# Autodesk Inventor assembly: Araknid-4Wire-Laser-Slot-x4
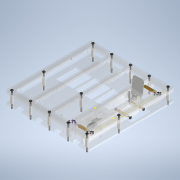
[picture p0: Inventor's stored thumbnail of the model, 180x180]
Saved by Autodesk Inventor 2021 (Build 250183000, 183)
## iProperties
Created: 2020-06-23
Part Number: Araknid-4Wire-Laser-Slot-x4
Document SubType Name: Assembly
Designer: lucas
Project: 4Wire-Laser
Author: lucas
Revision Number: RLS_001
## Documents named in this file (22)
- C:\Users\lucas\Nextcloud\HackerSpace\HV Home Battery Storage Project\Concepts & Storyboards\18650 4wire Holder\Araknid-4Wire-Laser-Slot-x4.iam
- C:\Users\lucas\Nextcloud\HackerSpace\HV Home Battery Storage Project\Concepts & Storyboards\18650 4wire Holder\4Wire-Laser-Slot\Laser-Slot-Term-Beam.ipt
- C:\Users\lucas\Nextcloud\HackerSpace\HV Home Battery Storage Project\Concepts & Storyboards\18650 4wire Holder\4Wire-Laser-Slot\Laser-Slot-Side.ipt
- C:\Users\lucas\Nextcloud\HackerSpace\HV Home Battery Storage Project\Concepts & Storyboards\18650 4wire Holder\4Wire-Laser-Slot\Laser-Slot-Bottom.ipt
- C:\Users\lucas\Nextcloud\HackerSpace\HV Home Battery Storage Project\Concepts & Storyboards\18650 4wire Holder\4Wire-Laser-Slot\Laser-Pivot-Term-Beam.ipt
- C:\Users\lucas\Nextcloud\HackerSpace\HV Home Battery Storage Project\Concepts & Storyboards\18650 4wire Holder\4Wire-Laser-Slot\Laser-Pivot-Side.ipt
- C:\Users\lucas\Nextcloud\HackerSpace\HV Home Battery Storage Project\Concepts & Storyboards\18650 4wire Holder\4Wire-Laser-Slot\Laser-Slot-Side_Mirror.ipt
- C:\Users\lucas\Nextcloud\HackerSpace\HV Home Battery Storage Project\Concepts & Storyboards\18650 4wire Holder\4Wire-Laser-Slot\Standoff-M3x26mm.ipt
- C:\Users\lucas\Nextcloud\HackerSpace\HV Home Battery Storage Project\Concepts & Storyboards\18650 4wire Holder\4Wire-Laser-Slot\Shaft5.ipt
- C:\Users\lucas\Nextcloud\HackerSpace\HV Home Battery Storage Project\Concepts & Storyboards\18650 4wire Holder\4Wire-Laser-Slot\Standoff-M3x20mm.ipt
- C:\Users\lucas\Nextcloud\HackerSpace\HV Home Battery Storage Project\Concepts & Storyboards\18650 4wire Holder\4Wire-Laser-Slot\Shaft7.ipt
- C:\Users\lucas\Nextcloud\HackerSpace\HV Home Battery Storage Project\Concepts & Storyboards\18650 4wire Holder\ZKE\ZKE-Term-Solid.ipt
- C:\Users\lucas\Nextcloud\HackerSpace\HV Home Battery Storage Project\Concepts & Storyboards\18650 4wire Holder\4Wire-Laser-Slot\Laser-Base-x4.ipt
- C:\Users\lucas\Nextcloud\HackerSpace\HV Home Battery Storage Project\Concepts & Storyboards\18650 4wire Holder\4Wire-Laser-Slot\Laser-Pivot-Ringpull.ipt
- C:\Users\lucas\Nextcloud\HackerSpace\HV Home Battery Storage Project\Concepts & Storyboards\18650 4wire Holder\4Wire-Laser-Slot\Laser-Slot-Endstop.ipt
- C:\Users\lucas\Nextcloud\HackerSpace\HV Home Battery Storage Project\Concepts & Storyboards\18650 4wire Holder\ZKE\ZKE-Term-Sprung.ipt
- C:\Users\lucas\Nextcloud\HackerSpace\HV Home Battery Storage Project\Concepts & Storyboards\18650 4wire Holder\ZKE\ZKE-Term-Solid-Shim.ipt
- C:\Users\lucas\Nextcloud\HackerSpace\HV Home Battery Storage Project\Concepts & Storyboards\18650 4wire Holder\4Wire-Laser-Slot\Laser-Slot-Top.ipt
- C:\Users\lucas\Nextcloud\HackerSpace\HV Home Battery Storage Project\Concepts & Storyboards\18650 4wire Holder\4Wire-Laser-Slot\Standoff-TH-M3x17mm.ipt
- C:\Users\lucas\Documents\Inventor\Content Center Files\R2021\en-US\ISO 7380-1\ISO 7380-1 - M3 x 10.ipt
- C:\Users\lucas\Documents\Inventor\Content Center Files\R2021\en-US\ISO 7380-1\ISO 7380-1 - M3 x 12.ipt
- C:\Users\lucas\Documents\Inventor\Content Center Files\R2021\en-US\ISO 4762(2)\ISO 4762 - M3 x 10ISO.ipt
## Components (52 placed, 17 different names)
1. PosTerminalBeamr:1 — Mate:24, Flush:6, Flush:10, Mate:38, Mate:39, Rotational:3
2. Laser-Slot-Side:2 — Flush:1, Mate:24, Flush:6, Mate:27, Flush:8, Mate:34, Mate:35, Flush:11, Flush:12, Mate:46, Mate:47, Flush:17, Mate:49, Mate:52, Mate:53
3. Laser-Slot-Endstop:1 — Mate:46, Mate:47, Flush:17
4. Laser-Slot-Bottom:1 — Mate:51, Mate:52, Mate:53
5. ZKE-Term-Sprung:1 — Rotational:3
6. Laser-Pivot-Term-Beam:1 — Mate:6, Mate:10, Flush:2, Flush:3, Mate:48, Rotational:5, Rotational:6, Rotational:7
7. Laser-Pivot-Side:1 — Mate:10, Flush:2, Mate:44, Flush:13, Angle:4, Mate:45, Flush:14, Angle:5, Flush:16
8. Laser-Pivot-Side:2 — Mate:6, Flush:3, Rotational:4, Rotation:1, Flush:16, Mate:48
9. Laser-Slot-Side_Mirror:1 — Mate:4, Mate:26, Flush:7, Mate:32, Mate:33, Flush:10, Mate:38, Mate:39, Flush:11, Flush:12, Rotational:1, Rotation:1, Mate:50, Mate:51
10. Shaft:1 — Mate:44, Flush:13, Angle:4
11. Shaft:1 — Mate:45, Flush:14, Angle:5
12. ISO 4762 M3 x 10:1
13. ISO 4762 M3 x 10:2
14. ISO 7380-1 M3 x 10:3
15. ISO 7380-1 M3 x 10:4
16. Shaft:1 — Mate:26, Flush:7
17. Shaft:1 — Mate:27, Flush:8
18. ISO 4762 M3 x 10:3
19. ISO 4762 M3 x 10:4
20. ISO 7380-1 M3 x 10:1 — Mate:32, Mate:33
21. ISO 7380-1 M3 x 10:2 — Mate:34, Mate:35
22. ZKE-Term-Solid:1 — Rotational:7
23. Laser-Base-x4:1 — Rotational:1, Rotational:4, Rotational:8, Rotational:9, Rotational:10, Rotational:11, Rigid:1, Rotational:12, Rotational:13, Rotational:14, Rotational:15, Rotational:16, Rotational:17, Rigid:2, Rotational:18, Mate:54, Mate:55, Mate:56, Mate:57, Mate:58, Mate:59, Mate:60, Mate:61, Mate:62, Mate:63, Mate:64, Mate:65, Mate:66, Mate:67, Mate:68, Mate:69, Mate:70, Mate:71, Mate:72, Mate:73, Mate:74, Mate:75, Mate:76, Mate:77, Mate:78, Mate:79
24. Laser-Pivot-Ringpull:1 — Rotational:5
25. ZKE-Term-Solid-Shim:1 — Rotational:6
26. Laser-Slot-Top:1 — Mate:49, Mate:50
27. Shaft:1 — Rotational:8
28. Shaft:2 — Rotational:10
29. Shaft:3 — Rotational:9
30. Shaft:4 — Rotational:11
31. Shaft:5 — Rigid:1
32. Shaft:6 — Rotational:16
33. Shaft:7 — Rotational:14
34. Shaft:8 — Rotational:15
35. Shaft:9 — Rotational:13
36. Shaft:10 — Rotational:12
37. Shaft:11 — Rotational:18
38. Shaft:12 — Rigid:2
39. Shaft:13 — Rotational:17
40. ISO 7380-1 M3 x 12:3 — Mate:54, Mate:55
41. ISO 7380-1 M3 x 12:4 — Mate:56, Mate:57
42. ISO 7380-1 M3 x 12:5 — Mate:58, Mate:59
43. ISO 7380-1 M3 x 12:6 — Mate:60, Mate:61
44. ISO 7380-1 M3 x 12:7 — Mate:62, Mate:63
45. ISO 7380-1 M3 x 12:8 — Mate:64, Mate:65
46. ISO 7380-1 M3 x 12:9 — Mate:66, Mate:67
47. ISO 7380-1 M3 x 12:10 — Mate:68, Mate:69
48. ISO 7380-1 M3 x 12:11 — Mate:70, Mate:71
49. ISO 7380-1 M3 x 12:12 — Mate:72, Mate:73
50. ISO 7380-1 M3 x 12:13 — Mate:74, Mate:75
51. ISO 7380-1 M3 x 12:14 — Mate:76, Mate:77
52. ISO 7380-1 M3 x 12:15 — Mate:78, Mate:79
## Relationships (95: Mate 60, RevoluteJoint 17, Flush 13, Angle 2, WeldJoint 2, RelateRotation 1)
- Flush:1 (10 mm): Laser-Slot-Side:2
- Mate:4 (10 mm): Laser-Slot-Side_Mirror:1
- Mate:6 (0.075 mm): Laser-Pivot-Term-Beam:1 ↔ Laser-Pivot-Side:2
- Mate:10 (0.075 mm): Laser-Pivot-Term-Beam:1 ↔ Laser-Pivot-Side:1
- Flush:2: Laser-Pivot-Term-Beam:1 ↔ Laser-Pivot-Side:1
- Flush:3: Laser-Pivot-Term-Beam:1 ↔ Laser-Pivot-Side:2
- [Mate]: Shaft:1 ↔ ISO 4762 M3 x 10:1
- [Mate]: Laser-Pivot-Side:1 ↔ ISO 4762 M3 x 10:1
- [Mate]: Shaft:1 ↔ ISO 4762 M3 x 10:2
- [Mate]: Laser-Pivot-Side:2 ↔ ISO 4762 M3 x 10:2
- [Mate]: Laser-Pivot-Side:1 ↔ ISO 7380-1 M3 x 10:3
- [Mate]: Laser-Pivot-Side:1 ↔ ISO 7380-1 M3 x 10:3
- [Mate]: Laser-Pivot-Side:2 ↔ ISO 7380-1 M3 x 10:4
- [Mate]: Laser-Pivot-Side:2 ↔ ISO 7380-1 M3 x 10:4
- Mate:24 (0.075 mm): PosTerminalBeamr:1 ↔ Laser-Slot-Side:2
- Flush:6: PosTerminalBeamr:1 ↔ Laser-Slot-Side:2
- Mate:26: Laser-Slot-Side_Mirror:1 ↔ Shaft:1
- Flush:7: Laser-Slot-Side_Mirror:1 ↔ Shaft:1
- Mate:27: Laser-Slot-Side:2 ↔ Shaft:1
- Flush:8: Laser-Slot-Side:2 ↔ Shaft:1
- [Mate]: Laser-Slot-Side:2 ↔ ISO 4762 M3 x 10:3
- [Mate]: Laser-Slot-Side:2 ↔ ISO 4762 M3 x 10:3
- [Mate]: Laser-Slot-Side_Mirror:1 ↔ ISO 4762 M3 x 10:4
- [Mate]: Laser-Slot-Side_Mirror:1 ↔ ISO 4762 M3 x 10:4
- Mate:32: Laser-Slot-Side_Mirror:1 ↔ ISO 7380-1 M3 x 10:1
- Mate:33: Laser-Slot-Side_Mirror:1 ↔ ISO 7380-1 M3 x 10:1
- Mate:34: Laser-Slot-Side:2 ↔ ISO 7380-1 M3 x 10:2
- Mate:35: Laser-Slot-Side:2 ↔ ISO 7380-1 M3 x 10:2
- Rotational:1 [RevoluteJoint] (1 mm): Laser-Slot-Side_Mirror:1 ↔ Laser-Base-x4:1
- Flush:10: PosTerminalBeamr:1 ↔ Laser-Slot-Side_Mirror:1
- Mate:38 (0.075 mm): PosTerminalBeamr:1 ↔ Laser-Slot-Side_Mirror:1
- Mate:39 (0.075 mm): PosTerminalBeamr:1 ↔ Laser-Slot-Side_Mirror:1
- Flush:11: Laser-Slot-Side:2 ↔ Laser-Slot-Side_Mirror:1
- Flush:12: Laser-Slot-Side:2 ↔ Laser-Slot-Side_Mirror:1
- Rotational:3 [RevoluteJoint]: PosTerminalBeamr:1 ↔ ZKE-Term-Sprung:1
- Rotational:4 [RevoluteJoint] (1 mm): Laser-Pivot-Side:2 ↔ Laser-Base-x4:1
- Rotation:1 [RelateRotation] (2.55 ul): Laser-Pivot-Side:2 ↔ Laser-Slot-Side_Mirror:1
- Mate:44: Laser-Pivot-Side:1 ↔ Shaft:1
- Flush:13: Laser-Pivot-Side:1 ↔ Shaft:1
- Angle:4 (0 deg): Laser-Pivot-Side:1 ↔ Shaft:1
- Mate:45: Laser-Pivot-Side:1 ↔ Shaft:1
- Flush:14: Laser-Pivot-Side:1 ↔ Shaft:1
- Angle:5 (0 deg): Laser-Pivot-Side:1 ↔ Shaft:1
- Mate:46: Laser-Slot-Side:2 ↔ Laser-Slot-Endstop:1
- Mate:47: Laser-Slot-Side:2 ↔ Laser-Slot-Endstop:1
- Flush:16: Laser-Pivot-Side:1 ↔ Laser-Pivot-Side:2
- Mate:48: Laser-Pivot-Term-Beam:1 ↔ Laser-Pivot-Side:2
- Flush:17 (2.75 mm): Laser-Slot-Side:2 ↔ Laser-Slot-Endstop:1
- Rotational:5 [RevoluteJoint]: Laser-Pivot-Term-Beam:1 ↔ Laser-Pivot-Ringpull:1
- Rotational:6 [RevoluteJoint]: Laser-Pivot-Term-Beam:1 ↔ ZKE-Term-Solid-Shim:1
- Rotational:7 [RevoluteJoint]: Laser-Pivot-Term-Beam:1 ↔ ZKE-Term-Solid:1
- Mate:49: Laser-Slot-Side:2 ↔ Laser-Slot-Top:1
- Mate:50: Laser-Slot-Side_Mirror:1 ↔ Laser-Slot-Top:1
- Mate:51: Laser-Slot-Bottom:1 ↔ Laser-Slot-Side_Mirror:1
- Mate:52: Laser-Slot-Side:2 ↔ Laser-Slot-Bottom:1
- Mate:53 (0.0375 mm): Laser-Slot-Side:2 ↔ Laser-Slot-Bottom:1
- Rotational:8 [RevoluteJoint]: Laser-Base-x4:1 ↔ Shaft:1
- Rotational:9 [RevoluteJoint]: Laser-Base-x4:1 ↔ Shaft:3
- Rotational:10 [RevoluteJoint]: Laser-Base-x4:1 ↔ Shaft:2
- Rotational:11 [RevoluteJoint]: Laser-Base-x4:1 ↔ Shaft:4
- Rigid:1 [WeldJoint]: Laser-Base-x4:1 ↔ Shaft:5
- Rotational:12 [RevoluteJoint]: Laser-Base-x4:1 ↔ Shaft:10
- Rotational:13 [RevoluteJoint]: Laser-Base-x4:1 ↔ Shaft:9
- Rotational:14 [RevoluteJoint]: Laser-Base-x4:1 ↔ Shaft:7
- Rotational:15 [RevoluteJoint]: Laser-Base-x4:1 ↔ Shaft:8
- Rotational:16 [RevoluteJoint]: Laser-Base-x4:1 ↔ Shaft:6
- Rotational:17 [RevoluteJoint]: Laser-Base-x4:1 ↔ Shaft:13
- Rigid:2 [WeldJoint]: Laser-Base-x4:1 ↔ Shaft:12
- Rotational:18 [RevoluteJoint]: Laser-Base-x4:1 ↔ Shaft:11
- Mate:54: Laser-Base-x4:1 ↔ ISO 7380-1 M3 x 12:3
- Mate:55: Laser-Base-x4:1 ↔ ISO 7380-1 M3 x 12:3
- Mate:56: Laser-Base-x4:1 ↔ ISO 7380-1 M3 x 12:4
- Mate:57: Laser-Base-x4:1 ↔ ISO 7380-1 M3 x 12:4
- Mate:58: Laser-Base-x4:1 ↔ ISO 7380-1 M3 x 12:5
- Mate:59: Laser-Base-x4:1 ↔ ISO 7380-1 M3 x 12:5
- Mate:60: Laser-Base-x4:1 ↔ ISO 7380-1 M3 x 12:6
- Mate:61: Laser-Base-x4:1 ↔ ISO 7380-1 M3 x 12:6
- Mate:62: Laser-Base-x4:1 ↔ ISO 7380-1 M3 x 12:7
- Mate:63: Laser-Base-x4:1 ↔ ISO 7380-1 M3 x 12:7
- Mate:64: Laser-Base-x4:1 ↔ ISO 7380-1 M3 x 12:8
- Mate:65: Laser-Base-x4:1 ↔ ISO 7380-1 M3 x 12:8
- Mate:66: Laser-Base-x4:1 ↔ ISO 7380-1 M3 x 12:9
- Mate:67: Laser-Base-x4:1 ↔ ISO 7380-1 M3 x 12:9
- Mate:68: Laser-Base-x4:1 ↔ ISO 7380-1 M3 x 12:10
- Mate:69: Laser-Base-x4:1 ↔ ISO 7380-1 M3 x 12:10
- Mate:70: Laser-Base-x4:1 ↔ ISO 7380-1 M3 x 12:11
- Mate:71: Laser-Base-x4:1 ↔ ISO 7380-1 M3 x 12:11
- Mate:72: Laser-Base-x4:1 ↔ ISO 7380-1 M3 x 12:12
- Mate:73: Laser-Base-x4:1 ↔ ISO 7380-1 M3 x 12:12
- Mate:74: Laser-Base-x4:1 ↔ ISO 7380-1 M3 x 12:13
- Mate:75: Laser-Base-x4:1 ↔ ISO 7380-1 M3 x 12:13
- Mate:76: Laser-Base-x4:1 ↔ ISO 7380-1 M3 x 12:14
- Mate:77: Laser-Base-x4:1 ↔ ISO 7380-1 M3 x 12:14
- Mate:78: Laser-Base-x4:1 ↔ ISO 7380-1 M3 x 12:15
- Mate:79: Laser-Base-x4:1 ↔ ISO 7380-1 M3 x 12:15
